# Autodesk Inventor assembly: Sortierer
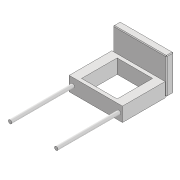
[picture p0: Inventor's stored thumbnail of the model, 180x180]
Saved by Autodesk Inventor 2020 (Build 240168000, 168)
## iProperties
Created: 2020-03-18
Part Number: Sortierer
Document SubType Name: Assembly
Designer: franz
Author: franz
## Documents named in this file (3)
- E:\Privat\Projekte\SPS_Training\Unity_SPS_Simulation\Unity_SPS_Schrittkette\CAD\Foerderband_V1\Sortierer\Sortierer.iam
- E:\Privat\Projekte\SPS_Training\Unity_SPS_Simulation\Unity_SPS_Schrittkette\CAD\Foerderband_V1\Sortierer\Grundkoerper.ipt
- E:\Privat\Projekte\SPS_Training\Unity_SPS_Simulation\Unity_SPS_Schrittkette\CAD\Foerderband_V1\Sortierer\Hubkolben.ipt
## Components (2 placed, 2 different names)
1. Grundkoerper:1 — Passend:1, Passend:2
2. Hubkolben:1 — Passend:1, Passend:2
## Relationships (2: Mate 2)
- Passend:1 [Mate]: Grundkoerper:1 ↔ Hubkolben:1
- Passend:2 [Mate]: Grundkoerper:1 ↔ Hubkolben:1
